# Autodesk Inventor assembly: BottleHolderV4Assembly
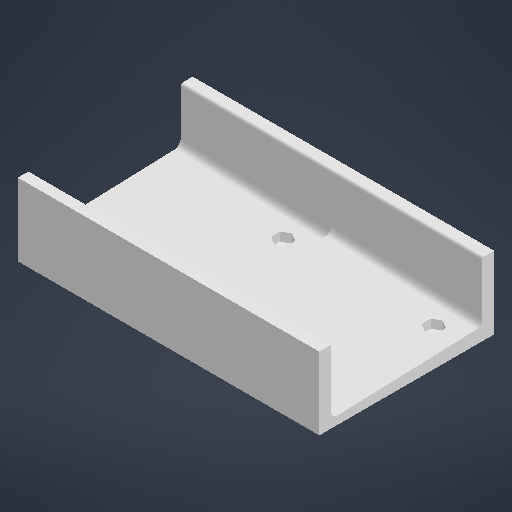
[picture p0: Inventor's stored thumbnail of the model, 512x512]
Saved by Autodesk Inventor 2025.1 (Build 291241020, 241B)
## iProperties
Created: 2025-05-04
Part Number: BottleHolderV4Assembly
Document SubType Name: Assembly
Designer: dpseu
Author: dpseu
## Documents named in this file (2)
- C:\Users\dpseu\workspace\Drink Table CAD Files\BottleHolderDoubleV1Assembly.iam
- C:\Users\dpseu\workspace\Drink Table CAD Files\BottleHolderDoubleV1.ipt
## Components (2 placed, 1 different names)
1. BottleHolderDoubleV1:1 — Mate:1, Flush:1, Flush:2
2. BottleHolderDoubleV1:2 — Mate:1, Flush:1, Flush:2
## Relationships (3: Flush 2, Mate 1)
- Mate:1: BottleHolderDoubleV1:1 ↔ BottleHolderDoubleV1:2
- Flush:1: BottleHolderDoubleV1:1 ↔ BottleHolderDoubleV1:2
- Flush:2: BottleHolderDoubleV1:1 ↔ BottleHolderDoubleV1:2
